# Autodesk Inventor assembly: 6_ Traction Tire - 0.5_ Wide (217-2860)
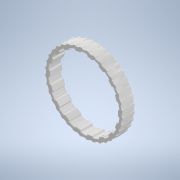
[picture p0: Inventor's stored thumbnail of the model, 180x180]
Saved by Autodesk Inventor 2021 (Build 250183000, 183)
## iProperties
Created: 2013-12-10
Part Number: 6_ Traction Tire - 0.5_ Wide (217-2860)
Description: STEP AP214
Document SubType Name: Assembly
Designer: con_c_000
Sending System: SolidWorks 2013
Preprocessor: SwSTEP 2.0
Title: 217-2860-STEP.STEP
Revision Number: ANY
## Documents named in this file (3)
- C:\Users\con_c_000\Documents\GitHub\RoboticsCad1111\PHRC CADD\Resources\VEXpro Resources\Wheels\Wheel Parts\6_ Traction Tire - 0.5_ Wide (217-2860).iam
- C:\Users\con_c_000\Documents\GitHub\RoboticsCad1111\PHRC CADD\Resources\VEXpro Resources\Wheels\Wheel Parts\217-2860-001 Rev3.ipt
- C:\Users\con_c_000\Documents\GitHub\RoboticsCad1111\PHRC CADD\Resources\VEXpro Resources\Wheels\Wheel Parts\217-2860-011 Rev1.ipt
## Components (2 placed, 2 different names)
1. 217-2860-001 Rev3_1 — Insert:1, Mate:1
2. 217-2860-011 Rev1_2 — Insert:1, Mate:1
## Relationships (2: Insert 1, Mate 1)
- Insert:1: 217-2860-001 Rev3_1 ↔ 217-2860-011 Rev1_2
- Mate:1: 217-2860-001 Rev3_1 ↔ 217-2860-011 Rev1_2
